# Autodesk Inventor assembly: Trail_assembly
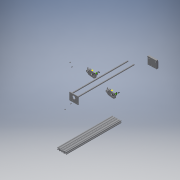
[picture p0: Inventor's stored thumbnail of the model, 180x180]
Saved by Autodesk Inventor 2019 (Build 230136000, 136)
## iProperties
Created: 2021-06-18
Part Number: Trail_assembly
Document SubType Name: Assembly
Designer: 91742
Author: 91742
## Documents named in this file (8)
- C:\Users\91742\3D Objects\Trail_assembly.iam
- C:\Users\91742\3D Objects\Rail_finished.ipt
- C:\Users\91742\3D Objects\Stepper_to_rail.ipt
- C:\Users\91742\3D Objects\Side_rod.ipt
- C:\Users\91742\3D Objects\Middle_part.ipt
- C:\Users\91742\3D Objects\Linear_ballbearing.ipt
- C:\Users\91742\3D Objects\End_atrail.ipt
- C:\Users\91742\3D Objects\Steeper nut.ipt
## Components (16 placed, 7 different names)
1. Rail_finished:1 — Rigid:1, Mate:1, Mate:2, Rotation:1, Insert:6
2. Rail_finished:2 — Rigid:1, Insert:5
3. Stepper_to_rail:1 — Mate:1, Mate:2, Rotation:1, Mate:3, Mate:4, Flush:2, Insert:5, Insert:6, Insert:7, Insert:8, Insert:10
4. Side_rod:1 — Flush:1, Mate:4, Insert:8
5. Side_rod:2 — Flush:1, Mate:3, Flush:2, Insert:7, Insert:10
6. Middle_part:1 — Insert:1, Insert:2
7. Middle_part:2 — Insert:3, Insert:4
8. Linear_ballbearing:1 — Insert:2
9. Linear_ballbearing:2 — Insert:1
10. Linear_ballbearing:3 — Insert:3
11. Linear_ballbearing:4 — Insert:4
12. End_atrail:1
13. Steeper nut:1
14. Steeper nut:2
15. Steeper nut:3
16. Steeper nut:4
## Relationships (17: Insert 9, Mate 4, Flush 2, WeldJoint 1, RelateRotation 1)
- Rigid:1 [WeldJoint]: Rail_finished:1 ↔ Rail_finished:2
- Mate:1: Rail_finished:1 ↔ Stepper_to_rail:1
- Mate:2: Rail_finished:1 ↔ Stepper_to_rail:1
- Rotation:1 [RelateRotation] (1 ul): Rail_finished:1 ↔ Stepper_to_rail:1
- Flush:1: Side_rod:1 ↔ Side_rod:2
- Mate:3: Stepper_to_rail:1 ↔ Side_rod:2
- Mate:4: Stepper_to_rail:1 ↔ Side_rod:1
- Flush:2: Stepper_to_rail:1 ↔ Side_rod:2
- Insert:1 (-16.5 mm): Middle_part:1 ↔ Linear_ballbearing:2
- Insert:2 (-16.5 mm): Middle_part:1 ↔ Linear_ballbearing:1
- Insert:3 (-16.5 mm): Middle_part:2 ↔ Linear_ballbearing:3
- Insert:4 (-16.5 mm): Middle_part:2 ↔ Linear_ballbearing:4
- Insert:5: Rail_finished:2 ↔ Stepper_to_rail:1
- Insert:6: Rail_finished:1 ↔ Stepper_to_rail:1
- Insert:7: Stepper_to_rail:1 ↔ Side_rod:2
- Insert:8: Stepper_to_rail:1 ↔ Side_rod:1
- Insert:10: Stepper_to_rail:1 ↔ Side_rod:2
